# Autodesk Inventor assembly: Leg_joint_roll_pitch
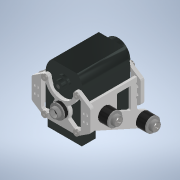
[picture p0: Inventor's stored thumbnail of the model, 180x180]
Saved by Autodesk Inventor 2020.4 (Build 244396000, 396)
## iProperties
Part Number: Leg_joint_roll_pitch
Document SubType Name: Assembly
Designer: Masato Kubotera
Mass: 155.537 g
Surface Area: 333.044 cm^2
Volume: 75.5065 cm^3
Density: 2.05992 g/cm^3
Author: Masato Kubotera
## Documents named in this file (17)
- C:\Users\Masato\Documents\Inventor\CIT Brains_Inventor\OpenPlatform_ver3_0（ワッシャ変更）\LowerBody\Leg_joit\Leg_joint_roll_pitch.iam
- C:\Users\Masato\Documents\Inventor\CIT Brains_Inventor\OpenPlatform_ver3_0（ワッシャ変更）\LowerBody\Leg_joit\Leg_joint_pitch_frame.ipt
- C:\Users\Masato\Documents\Inventor\CIT Brains_Inventor\OpenPlatform_ver3_0（ワッシャ変更）\LowerBody\Leg_joit\Leg_joint_roll_front_frame.ipt
- C:\Users\Masato\Documents\Inventor\CIT Brains_Inventor\OpenPlatform_ver3_0（ワッシャ変更）\Ready_Made\B3M11xx.ipt
- C:\Users\Masato\Documents\Inventor\CIT Brains_Inventor\OpenPlatform_ver3_0（ワッシャ変更）\Ready_Made\SLSBF6-39_5-M3-N3.ipt
- C:\Users\Masato\Documents\Inventor\CIT Brains_Inventor\OpenPlatform_ver3_0（ワッシャ変更）\Ready_Made\UUW-0312-10BH.ipt
- C:\Users\Masato\Documents\Inventor\CIT Brains_Inventor\OpenPlatform_ver3_0（ワッシャ変更）\Ready_Made\BRU-311S.ipt
- C:\Users\Masato\Documents\Inventor\CIT Brains_Inventor\OpenPlatform_ver3_0（ワッシャ変更）\Ready_Made\ARU-309S.ipt
- C:\Users\Masato\Documents\Inventor\CIT Brains_Inventor\OpenPlatform_ver3_0（ワッシャ変更）\Ready_Made\Screw\M3-6.ipt
- C:\Users\Masato\Documents\Inventor\CIT Brains_Inventor\OpenPlatform_ver3_0（ワッシャ変更）\Ready_Made\Screw\M2_6-20.ipt
- C:\Users\Masato\Documents\Inventor\CIT Brains_Inventor\OpenPlatform_ver3_0（ワッシャ変更）\Ready_Made\Screw\M2_6-15.ipt
- C:\Users\Masato\Documents\Inventor\CIT Brains_Inventor\OpenPlatform_ver3_0（ワッシャ変更）\Ready_Made\80F-0603.ipt
- C:\Users\Masato\Documents\Inventor\CIT Brains_Inventor\OpenPlatform_ver3_0（ワッシャ変更）\Ready_Made\CC-0612-15B.ipt
- C:\Users\Masato\Documents\Inventor\CIT Brains_Inventor\OpenPlatform_ver3_0（ワッシャ変更）\Ready_Made\CC-0612-50B.ipt
- C:\Users\Masato\Documents\Inventor\CIT Brains_Inventor\OpenPlatform_ver3_0（ワッシャ変更）\Ready_Made\SF319.ipt
- C:\Users\Masato\Documents\Inventor\CIT Brains_Inventor\OpenPlatform_ver3_0（ワッシャ変更）\Ready_Made\S3-07-3W.ipt
- C:\Users\Masato\Documents\Inventor\CIT Brains_Inventor\OpenPlatform_ver3_0（ワッシャ変更）\LowerBody\Leg_joit\Leg_joint_roll_frame.ipt
## Components (47 placed, 16 different names)
1. Leg_joint_pitch_frame:1 — メイト:2, フラッシュ:1, 挿入:11, 挿入:27, 挿入:28, 挿入:133
2. Leg_joint_pitch_frame:2 — メイト:3, メイト:4, フラッシュ:2, 挿入:12, 挿入:25, 挿入:26, フラッシュ:1, 挿入:132
3. Leg_joint_roll_front_frame:1 — 挿入:3, 挿入:4, 挿入:5, 挿入:6, メイト:2, メイト:3, メイト:4, フラッシュ:2, 挿入:81, 挿入:106, 挿入:107, 挿入:108, 挿入:109, 角度:1, 挿入:145
4. B3M11xx:1 — 挿入:3, 挿入:4, 挿入:5, 挿入:6, フラッシュ:6, メイト:8, メイト:10, 挿入:149, 挿入:150
5. SLSBF6-39_5-M3-N3:1 — 挿入:11, 挿入:12
6. UUW-0312-10BH:1 — 挿入:27, 挿入:100, 挿入:124
7. UUW-0312-10BH:2 — 挿入:28, 挿入:101, 挿入:125
8. UUW-0312-10BH:3 — 挿入:25, 挿入:99, 挿入:126
9. UUW-0312-10BH:4 — 挿入:26, 挿入:98, 挿入:127
10. UUW-0312-10BH:5 — 挿入:103, 挿入:121, 挿入:140
11. UUW-0312-10BH:6 — 挿入:81, 挿入:120
12. BRU-311S:1 — 挿入:99
13. BRU-311S:2 — 挿入:98
14. BRU-311S:3 — 挿入:101
15. BRU-311S:4 — 挿入:100
16. ARU-309S:2 — 挿入:103
17. M3-6:2 — 挿入:135
18. M2_6-20:1 — 挿入:106
19. M2_6-20:2 — 挿入:107
20. M2_6-20:3 — 挿入:108
21. M2_6-20:4 — 挿入:109
22. M2_6-15:1 — 挿入:141
23. M2_6-15:2 — 挿入:142
24. M2_6-15:3 — 挿入:143
25. M2_6-15:4 — 挿入:144
26. 80F-0603:1 — 挿入:134
27. 80F-0603:2 — 挿入:148
28. 80F-0603:3 — 挿入:130
29. 80F-0603:4 — 挿入:131
30. 80F-0603:5 — 挿入:129
31. 80F-0603:6 — 挿入:128
32. CC-0612-15B:1 — 挿入:114, 挿入:124
33. CC-0612-15B:2 — 挿入:115, 挿入:125
34. CC-0612-15B:3 — 挿入:116, 挿入:127
35. CC-0612-15B:4 — 挿入:117, 挿入:126
36. CC-0612-15B:5 — 挿入:120, 挿入:134
37. CC-0612-15B:6 — 挿入:121, 挿入:146
38. CC-0612-50B:1 — 挿入:114, 挿入:130
39. CC-0612-50B:2 — 挿入:115, 挿入:131
40. CC-0612-50B:3 — 挿入:116, 挿入:128
41. CC-0612-50B:4 — 挿入:117, 挿入:129
42. SF319:1 — 挿入:132
43. SF319:2 — 挿入:133
44. S3-07-3W:1 — 角度:1, 挿入:145
45. Leg_joint_roll_frame:1 — 挿入:135, 挿入:140, 挿入:141, 挿入:142, 挿入:143, 挿入:144, 挿入:149, 挿入:150
46. CC-0612-15B:7 — 挿入:146, 挿入:147
47. CC-0612-15B:8 — 挿入:147, 挿入:148
## Relationships (58: Insert 49, Mate 5, Flush 3, Angle 1)
- 挿入:3 [Insert]: Leg_joint_roll_front_frame:1 ↔ B3M11xx:1
- 挿入:4 [Insert]: Leg_joint_roll_front_frame:1 ↔ B3M11xx:1
- 挿入:5 [Insert]: Leg_joint_roll_front_frame:1 ↔ B3M11xx:1
- 挿入:6 [Insert]: Leg_joint_roll_front_frame:1 ↔ B3M11xx:1
- メイト:2 [Mate] (0.01 mm): Leg_joint_pitch_frame:1 ↔ Leg_joint_roll_front_frame:1
- フラッシュ:1 [Flush]: Leg_joint_pitch_frame:1 ↔ Leg_joint_pitch_frame:2
- メイト:3 [Mate] (0.01 mm): Leg_joint_pitch_frame:2 ↔ Leg_joint_roll_front_frame:1
- メイト:4 [Mate] (0.01 mm): Leg_joint_pitch_frame:2 ↔ Leg_joint_roll_front_frame:1
- フラッシュ:2 [Flush]: Leg_joint_pitch_frame:2 ↔ Leg_joint_roll_front_frame:1
- 挿入:11 [Insert]: Leg_joint_pitch_frame:1 ↔ SLSBF6-39_5-M3-N3:1
- 挿入:12 [Insert]: Leg_joint_pitch_frame:2 ↔ SLSBF6-39_5-M3-N3:1
- 挿入:25 [Insert]: Leg_joint_pitch_frame:2 ↔ UUW-0312-10BH:3
- 挿入:26 [Insert]: Leg_joint_pitch_frame:2 ↔ UUW-0312-10BH:4
- 挿入:27 [Insert]: Leg_joint_pitch_frame:1 ↔ UUW-0312-10BH:1
- 挿入:28 [Insert]: Leg_joint_pitch_frame:1 ↔ UUW-0312-10BH:2
- フラッシュ:6 [Flush]: B3M11xx:1
- メイト:8 [Mate]: B3M11xx:1
- メイト:10 [Mate]: B3M11xx:1
- 挿入:81 [Insert]: Leg_joint_roll_front_frame:1 ↔ UUW-0312-10BH:6
- 挿入:98 [Insert]: UUW-0312-10BH:4 ↔ BRU-311S:2
- 挿入:99 [Insert]: UUW-0312-10BH:3 ↔ BRU-311S:1
- 挿入:100 [Insert]: UUW-0312-10BH:1 ↔ BRU-311S:4
- 挿入:101 [Insert]: UUW-0312-10BH:2 ↔ BRU-311S:3
- 挿入:103 [Insert]: UUW-0312-10BH:5 ↔ ARU-309S:2
- 挿入:106 [Insert]: Leg_joint_roll_front_frame:1 ↔ M2_6-20:1
- 挿入:107 [Insert]: Leg_joint_roll_front_frame:1 ↔ M2_6-20:2
- 挿入:108 [Insert]: Leg_joint_roll_front_frame:1 ↔ M2_6-20:3
- 挿入:109 [Insert]: Leg_joint_roll_front_frame:1 ↔ M2_6-20:4
- 挿入:114 [Insert]: CC-0612-15B:1 ↔ CC-0612-50B:1
- 挿入:115 [Insert]: CC-0612-15B:2 ↔ CC-0612-50B:2
- 挿入:116 [Insert]: CC-0612-15B:3 ↔ CC-0612-50B:3
- 挿入:117 [Insert]: CC-0612-15B:4 ↔ CC-0612-50B:4
- 挿入:120 [Insert]: UUW-0312-10BH:6 ↔ CC-0612-15B:5
- 挿入:121 [Insert]: UUW-0312-10BH:5 ↔ CC-0612-15B:6
- 挿入:124 [Insert]: UUW-0312-10BH:1 ↔ CC-0612-15B:1
- 挿入:125 [Insert]: UUW-0312-10BH:2 ↔ CC-0612-15B:2
- 挿入:126 [Insert]: UUW-0312-10BH:3 ↔ CC-0612-15B:4
- 挿入:127 [Insert]: UUW-0312-10BH:4 ↔ CC-0612-15B:3
- 挿入:128 [Insert]: 80F-0603:6 ↔ CC-0612-50B:3
- 挿入:129 [Insert]: 80F-0603:5 ↔ CC-0612-50B:4
- 挿入:130 [Insert]: 80F-0603:3 ↔ CC-0612-50B:1
- 挿入:131 [Insert]: 80F-0603:4 ↔ CC-0612-50B:2
- 挿入:132 [Insert]: Leg_joint_pitch_frame:2 ↔ SF319:1
- 挿入:133 [Insert]: Leg_joint_pitch_frame:1 ↔ SF319:2
- 挿入:134 [Insert]: 80F-0603:1 ↔ CC-0612-15B:5
- 挿入:135 [Insert]: M3-6:2 ↔ Leg_joint_roll_frame:1
- 挿入:140 [Insert]: UUW-0312-10BH:5 ↔ Leg_joint_roll_frame:1
- 挿入:141 [Insert]: M2_6-15:1 ↔ Leg_joint_roll_frame:1
- 挿入:142 [Insert]: M2_6-15:2 ↔ Leg_joint_roll_frame:1
- 挿入:143 [Insert]: M2_6-15:3 ↔ Leg_joint_roll_frame:1
- 挿入:144 [Insert]: M2_6-15:4 ↔ Leg_joint_roll_frame:1
- 角度:1 [Angle] (0 deg): Leg_joint_roll_front_frame:1 ↔ S3-07-3W:1
- 挿入:145 [Insert]: Leg_joint_roll_front_frame:1 ↔ S3-07-3W:1
- 挿入:146 [Insert]: CC-0612-15B:6 ↔ CC-0612-15B:7
- 挿入:147 [Insert]: CC-0612-15B:7 ↔ CC-0612-15B:8
- 挿入:148 [Insert]: 80F-0603:2 ↔ CC-0612-15B:8
- 挿入:149 [Insert]: B3M11xx:1 ↔ Leg_joint_roll_frame:1
- 挿入:150 [Insert]: B3M11xx:1 ↔ Leg_joint_roll_frame:1
